# Autodesk Inventor assembly: Storage System Assembly
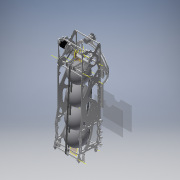
[picture p0: Inventor's stored thumbnail of the model, 180x180]
Saved by Autodesk Inventor 2019.4 (Build 234330000, 330)
## iProperties
Created: 2020-01-24
Part Number: Storage System Assembly
Document SubType Name: Assembly
Designer: admin
Mass: 7244.39 g
Surface Area: 20180.5 cm^2
Volume: 15125.5 cm^3
Density: 0.478951 g/cm^3
Author: admin
## Documents named in this file (35)
- C:\Users\admin\Desktop\FRC 2020 Engineering\GitHub\7738-2020\Robot V2\Storage System\Storage System Assembly.iam
- C:\Users\admin\Desktop\FRC 2020 Engineering\GitHub\7738-2020\Robot V2\Storage System\Storage Side Plate.ipt
- C:\Users\admin\Desktop\FRC 2020 Engineering\GitHub\7738-2020\Robot V2\Storage System\Storage System Assembly\Design Accelerator\Synchronous Belts Transmission1.iam
- C:\Users\admin\Desktop\FRC 2020 Engineering\GitHub\7738-2020\Robot V2\Storage System\Storage System Assembly\Design Accelerator\Synchronous Belts Transmission3.iam
- C:\Users\admin\Desktop\FRC 2020 Engineering\GitHub\7738-2020\Robot V2\Storage System\Storage System Assembly\Design Accelerator\Synchronous Belts Transmission4.iam
- C:\Users\admin\Desktop\FRC 2020 Engineering\GitHub\7738-2020\Robot V2\Storage System\Storage System Assembly\Design Accelerator\Synchronous Belts Transmission5.iam
- C:\Users\admin\Desktop\FRC 2020 Engineering\GitHub\7738-2020\Robot V2\Storage System\Storage System Assembly\Design Accelerator\Synchronous Belts Transmission6.iam
- C:\Users\admin\Desktop\FRC 2020 Engineering\GitHub\7738-2020\Power Cell.ipt
- C:\Users\admin\Desktop\FRC 2020 Engineering\GitHub\7738-2020\Robot V2\Storage System\Turret Support 2.ipt
- C:\Users\admin\Desktop\FRC 2020 Engineering\GitHub\7738-2020\Robot V2\Storage System\Turret Support.ipt
- C:\Users\admin\Desktop\FRC 2020 Engineering\GitHub\7738-2020\Robot V2\Storage System\Mounting Bracket.ipt
- C:\Users\admin\Desktop\FRC 2020 Engineering\GitHub\7738-2020\Robot V2\Storage System\Mounting Bracket 2.ipt
- C:\Users\admin\Desktop\FRC 2020 Engineering\GitHub\7738-2020\Robot V2\Storage System\Storage Plate Spacer.ipt
- C:\Users\admin\Desktop\FRC 2020 Engineering\GitHub\7738-2020\Robot V2\Storage System\Turret Bracket.ipt
- C:\Users\admin\Desktop\FRC 2020 Engineering\GitHub\7738-2020\Robot V2\Storage System\Small Support.ipt
- C:\Users\admin\Desktop\FRC 2020 Engineering\GitHub\7738-2020\Upper Stage\KFL08.ipt
- C:\Users\admin\Desktop\FRC 2020 Engineering\GitHub\7738-2020\Robot V2\Storage System\Turret Bracket 2.ipt
- C:\Users\admin\Desktop\FRC 2020 Engineering\GitHub\7738-2020\Robot V2\Storage System\Storage Axle.ipt
- C:\Users\admin\Desktop\FRC 2020 Engineering\GitHub\7738-2020\Robot V2\Storage System\Mini_CIM_Motor_217-3371.ipt
- C:\Users\admin\Desktop\FRC 2020 Engineering\GitHub\7738-2020\Robot V2\Storage System\Storage System Assembly\Design Accelerator\Synchronous Belts Transmission2.iam
- C:\Users\admin\Desktop\FRC 2020 Engineering\GitHub\7738-2020\Robot V2\Storage System\Motor Mount.ipt
- C:\Users\admin\Desktop\FRC 2020 Engineering\GitHub\7738-2020\Robot V2\Storage System\Motor Spacer.ipt
- C:\Users\admin\Desktop\FRC 2020 Engineering\GitHub\7738-2020\Elevator MK2\Wood Electronic  1.ipt
- C:\Users\admin\Desktop\FRC 2020 Engineering\GitHub\7738-2020\Robot V2\Turret\F6800.ipt
- C:\Users\admin\Desktop\FRC 2020 Engineering\GitHub\7738-2020\Robot V2\Storage System\Storage Axle Intake.ipt
- C:\Users\admin\Desktop\FRC 2020 Engineering\GitHub\7738-2020\Robot V2\Intake V2\Pneumatic Spcaer 2.ipt
- C:\Users\admin\Desktop\FRC 2020 Engineering\GitHub\7738-2020\Cover Spacer.ipt
- C:\Users\admin\Desktop\FRC 2020 Engineering\GitHub\7738-2020\Elevator MK2\Wood Electronic.ipt
- C:\Users\admin\Desktop\FRC 2020 Engineering\GitHub\7738-2020\Storage system\Back Ultrasonic sensor.ipt
- C:\Users\admin\Desktop\FRC 2020 Engineering\GitHub\7738-2020\Storage system\HC-SR04-UltrasonicSensor v7.ipt
- C:\Users\admin\Desktop\FRC 2020 Engineering\GitHub\7738-2020\Robot V2\Storage System\19_1 Chinesium.ipt
- C:\Users\admin\Desktop\FRC 2020 Engineering\GitHub\7738-2020\Robot V2\Storage System\3D printed Alternator\Inverter Assembly.iam
- C:\Users\admin\Desktop\FRC 2020 Engineering\GitHub\7738-2020\Robot V2\Storage System\Storage System Assembly\Design Accelerator\Synchronous Belts Transmission9.iam
- C:\Users\admin\Desktop\FRC 2020 Engineering\GitHub\7738-2020\Robot V2\Storage System\Storage System Assembly\Design Accelerator\Synchronous Belts Transmission10.iam
- C:\Users\admin\Desktop\FRC 2020 Engineering\GitHub\7738-2020\Robot V2\Storage System\Turret Driven Pinion.ipt
## Components (69 placed, 27 different names)
1. Storage Side Plate:1 — Mate:3, Flush:2, Mate:43, Mate:44, Mate:45, Mate:46, Mate:47, Mate:50, Mate:51, Mate:52, Flush:20, Mate:151, Mate:185, Mate:188, Mate:189, Mate:190, Mate:191, Mate:196, Mate:197, Mate:203, Mate:204, Flush:35, Mate:224, Mate:235, Flush:38, Mate:237, Flush:40, Mate:246, Mate:247, Mate:248, Mate:253, Mate:254, Mate:258, Mate:259, Mate:262, Flush:47, Mate:293, Mate:303, Flush:48, Angle:2, Mate:317, Mate:318, Mate:321, Mate:322, Mate:326, Mate:329, Mate:335, Mate:336, Mate:337
2. Synchronous Belts Transmission:1 [sub-assembly]
3. Synchronous Belts Transmission:2 [sub-assembly]
4. Synchronous Belts Transmission:3 [sub-assembly] — Symmetry:1
5. Synchronous Belts Transmission:4 [sub-assembly] — Symmetry:1
6. Synchronous Belts Transmission:5 [sub-assembly]
7. Power Cell:1 — Mate:4, Mate:231
8. Power Cell:2 — Mate:5, Mate:234
9. Power Cell:3 — Mate:6, Mate:232
10. Power Cell:4 — Mate:7, Mate:233
11. Mounting Bracket 2:1 — Mate:223, Flush:33
12. Mounting Bracket 2:2 — Mate:43, Flush:35
13. Storage Plate Spacer:1 — Mate:46, Mate:276
14. Storage Plate Spacer:3 — Mate:44, Mate:273
15. Storage Plate Spacer:4 — Mate:51, Mate:275
16. Storage Plate Spacer:5 — Mate:47, Mate:278
17. Storage Plate Spacer:6 — Mate:50, Mate:224
18. Storage Plate Spacer:8 — Mate:52, Mate:272
19. Storage Plate Spacer:9 — Mate:45, Mate:274
20. Turret Bracket:2 — Flush:25, Mate:169, Mate:283, Mate:287, Mate:288, Mate:300, Mate:301, Mate:309, Mate:334
21. Small Support:1 — Mate:304, Mate:305, Mate:308
22. Small Support:2 — Mate:283, Mate:300, Mate:301, Mate:302
23. Small Support:3 — Mate:287, Mate:288
24. Small Support:4 — Mate:306, Mate:307
25. Turret Support 2:2 — Mate:289, Mate:290, Flush:47, Mate:302, Mate:308, Mate:345, Mate:346, Mate:347, Mate:352
26. KFL08:2 — Mate:178, Mate:179, Mate:180, Mate:206
27. KFL08:3 — Mate:182, Mate:183, Mate:184, Mate:209
28. KFL08:4 — Mate:176, Mate:177, Mate:181, Mate:205
29. Turret Support:4 — Mate:289, Mate:290, Mate:293, Angle:1, Mate:323, Mate:324, Mate:325, Mate:327, Mate:328
30. Storage Side Plate:2 — Flush:20, Mate:151, Flush:25, Mate:169, Mate:176, Mate:177, Mate:178, Mate:179, Mate:180, Mate:181, Mate:182, Mate:183, Mate:184, Flush:27, Mate:214, Mate:215, Mate:216, Mate:223, Flush:33, Mate:236, Flush:39, Mate:244, Mate:245, Mate:249, Mate:252, Mate:255, Mate:268, Mate:272, Mate:273, Mate:274, Mate:275, Mate:276, Mate:278, Angle:1, Mate:315, Mate:316, Mate:319, Mate:320, Mate:330, Mate:334, Mate:348
31. KFL08:6 — Mate:188, Mate:196, Mate:197, Mate:200
32. KFL08:7 — Mate:189, Mate:190, Mate:191, Mate:202
33. KFL08:8 — Mate:185, Mate:201, Mate:203, Mate:204
34. Storage Axle:1 — Mate:202, Mate:206, Mate:349
35. Storage Axle:2 — Mate:201, Mate:205, Mate:350
36. Storage Axle:3 — Mate:200, Mate:209
37. Mini_CIM_Motor_217-3371:1 — Mate:210, Flush:27, Mate:211, Mate:212, Mate:213
38. Synchronous Belts Transmission:6 [sub-assembly] — Mate:210
39. Motor Mount:1 — Mate:211, Mate:212, Mate:213, Mate:214, Mate:217, Mate:218
40. Motor Spacer:1 — Mate:215, Mate:218
41. Motor Spacer:2 — Mate:216, Mate:217
42. Mounting Bracket:1 — Mate:235, Flush:38
43. Mounting Bracket:2 — Mate:236, Flush:39
44. Wood Electronic  1:1 — Mate:237, Flush:40, Mate:309, Mate:310, Mate:313, Mate:314
45. KFL08:9 — Mate:244, Mate:245, Mate:249, Mate:250
46. KFL08:10 — Mate:246, Mate:247, Mate:248, Mate:251
47. Storage Axle:4 — Mate:250, Mate:251
48. F6800:1 — Mate:252, Mate:255, Mate:256, Mate:257
49. F6800:2 — Mate:253, Mate:254
50. Storage Axle Intake:1 — Mate:256, Mate:257
51. Pneumatic Spcaer 2:1 — Mate:258, Mate:259
52. Cover Spacer:3 — Mate:262, Mate:329
53. Cover Spacer:4 — Mate:268, Mate:330
54. Turret Bracket:3 — Mate:303, Flush:48, Mate:304, Mate:305, Mate:306, Mate:307
55. Wood Electronic:1 — Mate:310, Mate:311, Mate:312, Mate:313
56. Wood Electronic:2 — Mate:311, Mate:312, Mate:314, Angle:2
57. Cover Spacer:7 — Mate:315, Mate:319
58. Cover Spacer:8 — Mate:316, Mate:320
59. Cover Spacer:9 — Mate:318, Mate:321
60. Cover Spacer:10 — Mate:317, Mate:322
61. Turret Bracket 2:3 — Mate:323, Mate:324, Mate:325
62. Turret Bracket 2:4 — Mate:326, Mate:327, Mate:328
63. Back Ultrasonic sensor:1 — Mate:335, Mate:336, Mate:337, Mate:338, Mate:339, Mate:340, Mate:343
64. HC-SR04-UltrasonicSensor v7:1 — Mate:338, Mate:343, Mate:344
65. 19_1 Chinesium:1 — Mate:345, Mate:346, Mate:347, Mate:351
66. Inverter Assembly:1 [sub-assembly] — Mate:348, Mate:349, Mate:350
67. Synchronous Belts Transmission:7 [sub-assembly]
68. Synchronous Belts Transmission:8 [sub-assembly]
69. Turret Driven Pinion:1 — Mate:351, Mate:352
## Relationships (151: Mate 137, Flush 11, Angle 2, Symmetry 1)
- Mate:3 (114.3 mm): Storage Side Plate:1
- Mate:4: Power Cell:1
- Mate:5: Power Cell:2
- Mate:6: Power Cell:3
- Mate:7: Power Cell:4
- Flush:2: Storage Side Plate:1
- Mate:43: Storage Side Plate:1 ↔ Mounting Bracket 2:2
- Mate:44: Storage Side Plate:1 ↔ Storage Plate Spacer:3
- Mate:45: Storage Side Plate:1 ↔ Storage Plate Spacer:9
- Mate:46: Storage Side Plate:1 ↔ Storage Plate Spacer:1
- Mate:47: Storage Side Plate:1 ↔ Storage Plate Spacer:5
- Mate:50: Storage Side Plate:1 ↔ Storage Plate Spacer:6
- Mate:51: Storage Side Plate:1 ↔ Storage Plate Spacer:4
- Mate:52: Storage Side Plate:1 ↔ Storage Plate Spacer:8
- Flush:20: Storage Side Plate:1 ↔ Storage Side Plate:2
- Mate:151 (228.6 mm): Storage Side Plate:1 ↔ Storage Side Plate:2
- Flush:25: Turret Bracket:2 ↔ Storage Side Plate:2
- Mate:169: Turret Bracket:2 ↔ Storage Side Plate:2
- Mate:176: KFL08:4 ↔ Storage Side Plate:2
- Mate:177: KFL08:4 ↔ Storage Side Plate:2
- Mate:178: KFL08:2 ↔ Storage Side Plate:2
- Mate:179: KFL08:2 ↔ Storage Side Plate:2
- Mate:180: KFL08:2 ↔ Storage Side Plate:2
- Mate:181: KFL08:4 ↔ Storage Side Plate:2
- Mate:182: KFL08:3 ↔ Storage Side Plate:2
- Mate:183: KFL08:3 ↔ Storage Side Plate:2
- Mate:184: KFL08:3 ↔ Storage Side Plate:2
- Mate:185: Storage Side Plate:1 ↔ KFL08:8
- Mate:188: Storage Side Plate:1 ↔ KFL08:6
- Mate:189: Storage Side Plate:1 ↔ KFL08:7
- Mate:190: Storage Side Plate:1 ↔ KFL08:7
- Mate:191: Storage Side Plate:1 ↔ KFL08:7
- Mate:196: Storage Side Plate:1 ↔ KFL08:6
- Mate:197: Storage Side Plate:1 ↔ KFL08:6
- Mate:200: KFL08:6 ↔ Storage Axle:3
- Mate:201: KFL08:8 ↔ Storage Axle:2
- Mate:202: KFL08:7 ↔ Storage Axle:1
- Mate:203: Storage Side Plate:1 ↔ KFL08:8
- Mate:204: Storage Side Plate:1 ↔ KFL08:8
- Mate:205: KFL08:4 ↔ Storage Axle:2
- Mate:206: KFL08:2 ↔ Storage Axle:1
- Mate:209: KFL08:3 ↔ Storage Axle:3
- Mate:210: Mini_CIM_Motor_217-3371:1 ↔ Synchronous Belts Transmission:6
- Flush:27 (-5 mm): Storage Side Plate:2 ↔ Mini_CIM_Motor_217-3371:1
- Mate:211: Mini_CIM_Motor_217-3371:1 ↔ Motor Mount:1
- Mate:212: Mini_CIM_Motor_217-3371:1 ↔ Motor Mount:1
- Mate:213: Mini_CIM_Motor_217-3371:1 ↔ Motor Mount:1
- Mate:214: Storage Side Plate:2 ↔ Motor Mount:1
- Mate:215: Storage Side Plate:2 ↔ Motor Spacer:1
- Mate:216: Storage Side Plate:2 ↔ Motor Spacer:2
- Mate:217: Motor Mount:1 ↔ Motor Spacer:2
- Mate:218: Motor Mount:1 ↔ Motor Spacer:1
- Mate:223: Mounting Bracket 2:1 ↔ Storage Side Plate:2
- Flush:33: Mounting Bracket 2:1 ↔ Storage Side Plate:2
- Flush:35: Storage Side Plate:1 ↔ Mounting Bracket 2:2
- Mate:224: Storage Side Plate:1 ↔ Storage Plate Spacer:6
- Symmetry:1: Synchronous Belts Transmission:3 ↔ Synchronous Belts Transmission:4
- Mate:231: Power Cell:1
- Mate:232: Power Cell:3
- Mate:233: Power Cell:4
- Mate:234: Power Cell:2
- Mate:235: Storage Side Plate:1 ↔ Mounting Bracket:1
- Mate:236: Storage Side Plate:2 ↔ Mounting Bracket:2
- Flush:38 (45 mm): Storage Side Plate:1 ↔ Mounting Bracket:1
- Flush:39 (45 mm): Storage Side Plate:2 ↔ Mounting Bracket:2
- Mate:237: Storage Side Plate:1 ↔ Wood Electronic  1:1
- Flush:40: Storage Side Plate:1 ↔ Wood Electronic  1:1
- Mate:244: Storage Side Plate:2 ↔ KFL08:9
- Mate:245: Storage Side Plate:2 ↔ KFL08:9
- Mate:246: Storage Side Plate:1 ↔ KFL08:10
- Mate:247: Storage Side Plate:1 ↔ KFL08:10
- Mate:248: Storage Side Plate:1 ↔ KFL08:10
- Mate:249: Storage Side Plate:2 ↔ KFL08:9
- Mate:250: KFL08:9 ↔ Storage Axle:4
- Mate:251: KFL08:10 ↔ Storage Axle:4
- Mate:252: Storage Side Plate:2 ↔ F6800:1
- Mate:253: Storage Side Plate:1 ↔ F6800:2
- Mate:254 (0.2 mm): Storage Side Plate:1 ↔ F6800:2
- Mate:255 (0.2 mm): Storage Side Plate:2 ↔ F6800:1
- Mate:256: F6800:1 ↔ Storage Axle Intake:1
- Mate:257: F6800:1 ↔ Storage Axle Intake:1
- Mate:258: Storage Side Plate:1 ↔ Pneumatic Spcaer 2:1
- Mate:259: Storage Side Plate:1 ↔ Pneumatic Spcaer 2:1
- Mate:262: Storage Side Plate:1 ↔ Cover Spacer:3
- Mate:268: Storage Side Plate:2 ↔ Cover Spacer:4
- Mate:272: Storage Plate Spacer:8 ↔ Storage Side Plate:2
- Mate:273: Storage Plate Spacer:3 ↔ Storage Side Plate:2
- Mate:274: Storage Plate Spacer:9 ↔ Storage Side Plate:2
- Mate:275: Storage Plate Spacer:4 ↔ Storage Side Plate:2
- Mate:276: Storage Plate Spacer:1 ↔ Storage Side Plate:2
- Mate:278: Storage Plate Spacer:5 ↔ Storage Side Plate:2
- Mate:283: Turret Bracket:2 ↔ Small Support:2
- Mate:287: Turret Bracket:2 ↔ Small Support:3
- Mate:288: Turret Bracket:2 ↔ Small Support:3
- Mate:289: Turret Support 2:2 ↔ Turret Support:4
- Mate:290 (15.4 mm): Turret Support 2:2 ↔ Turret Support:4
- Flush:47: Storage Side Plate:1 ↔ Turret Support 2:2
- Mate:293: Storage Side Plate:1 ↔ Turret Support:4
- Angle:1 (0 deg): Turret Support:4 ↔ Storage Side Plate:2
- Mate:300: Turret Bracket:2 ↔ Small Support:2
- Mate:301: Turret Bracket:2 ↔ Small Support:2
- Mate:302: Small Support:2 ↔ Turret Support 2:2
- Mate:303: Storage Side Plate:1 ↔ Turret Bracket:3
- Flush:48: Storage Side Plate:1 ↔ Turret Bracket:3
- Mate:304: Small Support:1 ↔ Turret Bracket:3
- Mate:305: Small Support:1 ↔ Turret Bracket:3
- Mate:306: Small Support:4 ↔ Turret Bracket:3
- Mate:307: Small Support:4 ↔ Turret Bracket:3
- Mate:308: Small Support:1 ↔ Turret Support 2:2
- Mate:309 (110 mm): Turret Bracket:2 ↔ Wood Electronic  1:1
- Mate:310: Wood Electronic  1:1 ↔ Wood Electronic:1
- Mate:311: Wood Electronic:1 ↔ Wood Electronic:2
- Mate:312: Wood Electronic:1 ↔ Wood Electronic:2
- Mate:313 (190 mm): Wood Electronic  1:1 ↔ Wood Electronic:1
- Mate:314 (275 mm): Wood Electronic  1:1 ↔ Wood Electronic:2
- Angle:2 (0 deg): Storage Side Plate:1 ↔ Wood Electronic:2
- Mate:315: Storage Side Plate:2 ↔ Cover Spacer:7
- Mate:316: Storage Side Plate:2 ↔ Cover Spacer:8
- Mate:317: Storage Side Plate:1 ↔ Cover Spacer:10
- Mate:318: Storage Side Plate:1 ↔ Cover Spacer:9
- Mate:319: Storage Side Plate:2 ↔ Cover Spacer:7
- Mate:320: Storage Side Plate:2 ↔ Cover Spacer:8
- Mate:321: Storage Side Plate:1 ↔ Cover Spacer:9
- Mate:322: Storage Side Plate:1 ↔ Cover Spacer:10
- Mate:323: Turret Support:4 ↔ Turret Bracket 2:3
- Mate:324: Turret Support:4 ↔ Turret Bracket 2:3
- Mate:325: Turret Support:4 ↔ Turret Bracket 2:3
- Mate:326: Storage Side Plate:1 ↔ Turret Bracket 2:4
- Mate:327: Turret Support:4 ↔ Turret Bracket 2:4
- Mate:328: Turret Support:4 ↔ Turret Bracket 2:4
- Mate:329: Storage Side Plate:1 ↔ Cover Spacer:3
- Mate:330: Storage Side Plate:2 ↔ Cover Spacer:4
- Mate:334: Turret Bracket:2 ↔ Storage Side Plate:2
- Mate:335: Storage Side Plate:1 ↔ Back Ultrasonic sensor:1
- Mate:336: Storage Side Plate:1 ↔ Back Ultrasonic sensor:1
- Mate:337: Storage Side Plate:1 ↔ Back Ultrasonic sensor:1
- Mate:338: Back Ultrasonic sensor:1 ↔ HC-SR04-UltrasonicSensor v7:1
- Mate:339: Back Ultrasonic sensor:1
- Mate:340: Back Ultrasonic sensor:1
- Mate:341
- Mate:342
- Mate:343: Back Ultrasonic sensor:1 ↔ HC-SR04-UltrasonicSensor v7:1
- Mate:344: HC-SR04-UltrasonicSensor v7:1
- Mate:345: Turret Support 2:2 ↔ 19_1 Chinesium:1
- Mate:346: Turret Support 2:2 ↔ 19_1 Chinesium:1
- Mate:347: Turret Support 2:2 ↔ 19_1 Chinesium:1
- Mate:348: Storage Side Plate:2 ↔ Inverter Assembly:1
- Mate:349 (45 mm): Storage Axle:1 ↔ Inverter Assembly:1
- Mate:350 (85 mm): Storage Axle:2 ↔ Inverter Assembly:1
- Mate:351: 19_1 Chinesium:1 ↔ Turret Driven Pinion:1
- Mate:352 (14.8 mm): Turret Support 2:2 ↔ Turret Driven Pinion:1
